# Autodesk Inventor assembly: RT_FRM_A_003_FrameV3
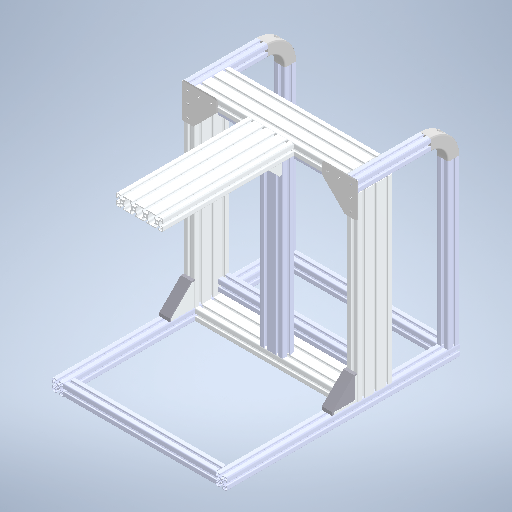
[picture p0: Inventor's stored thumbnail of the model, 512x512]
Saved by Autodesk Inventor 2025.3 (Build 293356000, 356)
## iProperties
Created: 2026-06-06
Part Number: RT_FRM_A_003_FrameV3
Document SubType Name: Assembly
Designer: louis
Author: louis
## Documents named in this file (14)
- C:\Users\louis\OneDrive\Desktop\R_Trident\02_CAD\04_Subassemblies\RT_FRM_A_003_FrameV3.iam
- C:\Users\louis\OneDrive\Desktop\R_Trident\02_CAD\01_Standard_Parts\02_FRM_Extrusions_Frame_V3\4040x700.ipt
- C:\Users\louis\OneDrive\Desktop\R_Trident\02_CAD\01_Standard_Parts\02_FRM_Extrusions_Frame_V3\40120x620.ipt
- C:\Users\louis\OneDrive\Desktop\R_Trident\02_CAD\01_Standard_Parts\02_FRM_Extrusions_Frame_V3\4040x300.ipt
- C:\Users\louis\OneDrive\Desktop\R_Trident\02_CAD\01_Standard_Parts\02_FRM_Extrusions_Frame_V3\40160x400.ipt
- C:\Users\louis\OneDrive\Desktop\R_Trident\02_CAD\01_Standard_Parts\02_FRM_Extrusions_Frame_V3\4080x600.ipt
- C:\Users\louis\OneDrive\Desktop\R_Trident\02_CAD\01_Standard_Parts\02_FRM_Extrusions_Frame_V3\4040x620.ipt
- C:\Users\louis\OneDrive\Desktop\R_Trident\02_CAD\03_Parts_Custom\RT_FRM_MC_013_R100_Door_Roundover.ipt
- C:\Users\louis\OneDrive\Desktop\R_Trident\02_CAD\01_Standard_Parts\02_FRM_Extrusions_Frame_V3\4040x560.ipt
- C:\Users\louis\OneDrive\Desktop\R_Trident\02_CAD\01_Standard_Parts\02_FRM_Extrusions_Frame_V3\40120x520.ipt
- C:\Users\louis\OneDrive\Desktop\R_Trident\02_CAD\01_Standard_Parts\03_FRM_Fastener\8080L\A_8080L.iam
- C:\Users\louis\OneDrive\Desktop\R_Trident\02_CAD\01_Standard_Parts\02_FRM_Extrusions_Frame_V3\4040xElectricalPannelSupport.ipt
- C:\Users\louis\OneDrive\Desktop\R_Trident\02_CAD\01_Standard_Parts\03_FRM_Fastener\Connection_plate_L_120x120.ipt
- C:\Users\louis\OneDrive\Desktop\R_Trident\02_CAD\01_Standard_Parts\03_FRM_Fastener\4080L\A_4080L.iam
## Components (23 placed, 13 different names)
1. 4040x700:1 — Mate:2, Mate:3, Flush:1, Flush:3, Flush:5, Flush:24, Flush:25, Flush:26, Mate:50, Flush:39, Mate:59, Flush:58
2. 40120x620:1 — Mate:1, Flush:4, Flush:6, Mate:5, Flush:10, Flush:15, Mate:6, Symmetry:1, Flush:56, Mate:58, Flush:57
3. 40120x520:1 — Flush:8, Mate:5, Flush:9, Flush:11, Mate:7, Flush:16, Symmetry:2, Symmetry:3, Flush:22, Flush:53, Flush:55
4. 40120x620:3 — Mate:3, Flush:3, Flush:6, Flush:7, Flush:8, Flush:12, Symmetry:1, Flush:24, Flush:27, Mate:53, Mate:54, Flush:51, Flush:52, Flush:54, Mate:60
5. 40120x520:2 — Mate:2, Mate:4, Flush:1, Flush:2, Flush:7, Mate:17, Symmetry:2, Symmetry:3
6. 4040x700:2 — Mate:1, Mate:4, Flush:2, Flush:4, Flush:5, Mate:25, Flush:38, Mate:51, Mate:61
7. 4040x300:1 — Flush:9, Flush:10, Flush:15, Mate:6, Mate:26, Mate:27, Mate:56
8. 4040x300:2 — Flush:11, Flush:12, Mate:30, Mate:31, Flush:27, Mate:57
9. 40160x400:1 — Mate:7, Flush:16, Mate:37, Flush:50
10. 4080x600:1 — Mate:17, Flush:22, Mate:36
11. 4040x620:1 — Mate:25, Flush:25, Flush:26
12. RT_FRM_MC_013_R100_Door_Roundover:1 — Mate:26, Mate:27, Mate:28, Mate:29
13. 4040x560:1 — Mate:28, Mate:29
14. 4040x560:2 — Mate:32, Mate:33
15. RT_FRM_MC_013_R100_Door_Roundover:2 — Mate:30, Mate:31, Mate:32, Mate:33
16. A_8080L:1 [sub-assembly] — Mate:36, Mate:37
17. 4040x620:2 — Flush:38, Mate:50, Mate:51, Flush:39
18. 4040xElectricalPannelSupport:1 — Mate:53, Flush:52, Mate:55, Symmetry:4
19. 4040xElectricalPannelSupport:2 — Mate:54, Flush:51, Mate:55, Symmetry:4
20. Connection_plate_L_120x120:1 — Flush:53, Flush:54, Mate:57
21. Connection_plate_L_120x120:2 — Flush:55, Flush:56, Mate:56
22. A_4080L:1 [sub-assembly] — Mate:58, Mate:61, Flush:57
23. A_4080L:2 [sub-assembly] — Mate:59, Mate:60, Flush:58
## Relationships (68: Mate 34, Flush 30, Symmetry 4)
- Mate:1: 40120x620:1 ↔ 4040x700:2
- Mate:2: 4040x700:1 ↔ 40120x520:2
- Mate:3: 4040x700:1 ↔ 40120x620:3
- Mate:4: 40120x520:2 ↔ 4040x700:2
- Flush:1: 4040x700:1 ↔ 40120x520:2
- Flush:2: 40120x520:2 ↔ 4040x700:2
- Flush:3: 4040x700:1 ↔ 40120x620:3
- Flush:4: 40120x620:1 ↔ 4040x700:2
- Flush:5: 4040x700:1 ↔ 4040x700:2
- Flush:6: 40120x620:1 ↔ 40120x620:3
- Flush:7: 40120x620:3 ↔ 40120x520:2
- Flush:8: 40120x520:1 ↔ 40120x620:3
- Mate:5: 40120x620:1 ↔ 40120x520:1
- Flush:9: 40120x520:1 ↔ 4040x300:1
- Flush:10: 40120x620:1 ↔ 4040x300:1
- Flush:11: 40120x520:1 ↔ 4040x300:2
- Flush:12: 40120x620:3 ↔ 4040x300:2
- Flush:15: 40120x620:1 ↔ 4040x300:1
- Mate:6: 40120x620:1 ↔ 4040x300:1
- Mate:7: 40120x520:1 ↔ 40160x400:1
- Flush:16: 40120x520:1 ↔ 40160x400:1
- Mate:17: 40120x520:2 ↔ 4080x600:1
- Symmetry:1: 40120x620:1 ↔ 40120x620:3
- Symmetry:2: 40120x520:1 ↔ 40120x520:2
- Symmetry:3: 40120x520:1 ↔ 40120x520:2
- Mate:19
- Mate:20
- Mate:21
- Flush:22: 40120x520:1 ↔ 4080x600:1
- Flush:24 (450 mm): 4040x700:1 ↔ 40120x620:3
- Mate:25: 4040x700:2 ↔ 4040x620:1
- Flush:25: 4040x700:1 ↔ 4040x620:1
- Flush:26: 4040x700:1 ↔ 4040x620:1
- Mate:26: 4040x300:1 ↔ RT_FRM_MC_013_R100_Door_Roundover:1
- Mate:27: 4040x300:1 ↔ RT_FRM_MC_013_R100_Door_Roundover:1
- Mate:28: RT_FRM_MC_013_R100_Door_Roundover:1 ↔ 4040x560:1
- Mate:29: RT_FRM_MC_013_R100_Door_Roundover:1 ↔ 4040x560:1
- Mate:30: 4040x300:2 ↔ RT_FRM_MC_013_R100_Door_Roundover:2
- Mate:31: 4040x300:2 ↔ RT_FRM_MC_013_R100_Door_Roundover:2
- Mate:32: 4040x560:2 ↔ RT_FRM_MC_013_R100_Door_Roundover:2
- Mate:33: 4040x560:2 ↔ RT_FRM_MC_013_R100_Door_Roundover:2
- Flush:27: 40120x620:3 ↔ 4040x300:2
- Mate:36: 4080x600:1 ↔ A_8080L:1
- Mate:37: 40160x400:1 ↔ A_8080L:1
- Flush:38: 4040x700:2 ↔ 4040x620:2
- Mate:50: 4040x700:1 ↔ 4040x620:2
- Mate:51: 4040x700:2 ↔ 4040x620:2
- Flush:39: 4040x700:1 ↔ 4040x620:2
- Flush:50: 40160x400:1
- Mate:53: 40120x620:3 ↔ 4040xElectricalPannelSupport:1
- Mate:54: 40120x620:3 ↔ 4040xElectricalPannelSupport:2
- Flush:51: 40120x620:3 ↔ 4040xElectricalPannelSupport:2
- Flush:52: 40120x620:3 ↔ 4040xElectricalPannelSupport:1
- Mate:55 (485 mm): 4040xElectricalPannelSupport:1 ↔ 4040xElectricalPannelSupport:2
- Flush:53: 40120x520:1 ↔ Connection_plate_L_120x120:1
- Flush:54: 40120x620:3 ↔ Connection_plate_L_120x120:1
- Flush:55: 40120x520:1 ↔ Connection_plate_L_120x120:2
- Flush:56: 40120x620:1 ↔ Connection_plate_L_120x120:2
- Mate:56: 4040x300:1 ↔ Connection_plate_L_120x120:2
- Mate:57: 4040x300:2 ↔ Connection_plate_L_120x120:1
- Mate:58: 40120x620:1 ↔ A_4080L:1
- Mate:59: 4040x700:1 ↔ A_4080L:2
- Mate:60: 40120x620:3 ↔ A_4080L:2
- Mate:61: 4040x700:2 ↔ A_4080L:1
- Flush:57 (3 mm): 40120x620:1 ↔ A_4080L:1
- Flush:58 (3 mm): 4040x700:1 ↔ A_4080L:2
- Symmetry:4: 4040xElectricalPannelSupport:1 ↔ 4040xElectricalPannelSupport:2
- Mate:63 (-20 mm)
